# Autodesk Inventor assembly: 組合1
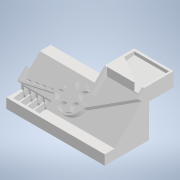
[picture p0: Inventor's stored thumbnail of the model, 180x180]
Saved by Autodesk Inventor 2020 (Build 240168000, 168)
## iProperties
Created: 2021-01-06
Part Number: 組合1
Document SubType Name: Assembly
Designer: User
Author: User
## Documents named in this file (3)
- C:\Users\User\Desktop\組合1.iam
- C:\Users\User\Desktop\github.ipt
- C:\Users\User\Desktop\零件2-1.ipt
## Components (2 placed, 2 different names)
1. github:1 — 貼合:1, 貼合:2
2. 零件2-1:1 — 貼合:1, 貼合:2
## Relationships (2: Mate 2)
- 貼合:1 [Mate]: github:1 ↔ 零件2-1:1
- 貼合:2 [Mate]: github:1 ↔ 零件2-1:1
